# Autodesk Inventor assembly: 42146-31
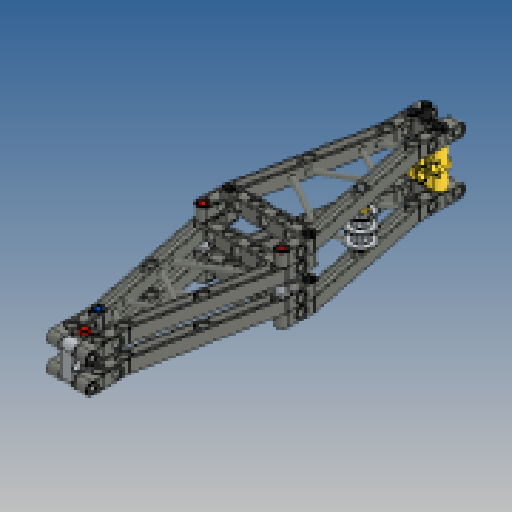
[picture p0: Inventor's stored thumbnail of the model, 512x512]
Saved by Autodesk Inventor 2025 (Build 290162010, 162A)
## iProperties
Created: 2024-12-05
Part Number: 42146-31
Material: Generisch
Document SubType Name: Assembly
Designer: hp.muther
Author: hp.muther
## Documents named in this file (15)
- D:\Inventor\Projekte\Muther\LEGO Technic\LEGO Technik - Raupenkran LR 13000 (42146)\42146-31.iam
- D:\Inventor\Projekte\Muther\LEGO Technic\LEGO Pieces\Rahmen, T-Stücke\79768-DkBluishGray.ipt
- D:\Inventor\Projekte\Muther\LEGO Technic\LEGO Pieces\Pin's\4274-Red.ipt
- D:\Inventor\Projekte\Muther\LEGO Technic\LEGO Pieces\Pin's\11214-Red.ipt
- D:\Inventor\Projekte\Muther\LEGO Technic\LEGO Pieces\Pin's\32054-LtBluishGray.ipt
- D:\Inventor\Projekte\Muther\LEGO Technic\LEGO Pieces\Pin's\2780-Black.ipt
- D:\Inventor\Projekte\Muther\LEGO Technic\LEGO Pieces\Achsen\32073-LtBluishGray.ipt
- D:\Inventor\Projekte\Muther\LEGO Technic\LEGO Pieces\Räder, Raupe\42610-LtBluishGray.ipt
- D:\Inventor\Projekte\Muther\LEGO Technic\LEGO Pieces\Pin's\6558-Blue.ipt
- D:\Inventor\Projekte\Muther\LEGO Technic\LEGO Pieces\Rund\18654-DkBluishGray.ipt
- D:\Inventor\Projekte\Muther\LEGO Technic\LEGO Pieces\Verbindungselemente\39793-Yellow.ipt
- D:\Inventor\Projekte\Muther\LEGO Technic\LEGO Pieces\Rund\4265c-Yellow.ipt
- D:\Inventor\Projekte\Muther\LEGO Technic\LEGO Pieces\Diverses\61510-LtBluishGray.ipt
- D:\Inventor\Projekte\Muther\LEGO Technic\LEGO Pieces\Pin's\77765-MediumStoneGrey.ipt
- D:\Inventor\Projekte\Muther\LEGO Technic\LEGO Pieces\Lochbalken\32523-LtBluishGray.ipt
## Components (32 placed, 14 different names)
1. 79768-DkBluishGray:1 — Einfügen:2, Einfügen:3, Einfügen:4, Einfügen:6, Einfügen:7, Einfügen:20, Einfügen:22, Einfügen:40, Einfügen:45
2. 4274-Red:1 — Einfügen:2
3. 11214-Red:1 — Einfügen:1, Passend:4
4. 32054-LtBluishGray:1 — Einfügen:1, Einfügen:7
5. 2780-Black:1 — Einfügen:3
6. 2780-Black:2 — Einfügen:4
7. 11214-Red:2
8. 32054-LtBluishGray:2 — Einfügen:6, Einfügen:26, Passend:8
9. 6558-Blue:1 — Einfügen:21, Einfügen:22
10. 18654-DkBluishGray:1 — Einfügen:21
11. 42610-LtBluishGray:4 — Einfügen:20
12. 79768-DkBluishGray:2 — Einfügen:26, Passend:4, Einfügen:34, Einfügen:43, Einfügen:44
13. 4274-Red:2
14. 2780-Black:3
15. 2780-Black:4 — Passend:7
16. 2780-Black:5
17. 2780-Black:6
18. 2780-Black:7 — Passend:6
19. 2780-Black:8
20. 39793-Yellow:1 — Einfügen:33
21. 79768-DkBluishGray:3 — Einfügen:33, Passend:6, Einfügen:34, Passend:7, Einfügen:39, Einfügen:41
22. 4265c-Yellow:1 — Einfügen:35, Fluchtend:1
23. 61510-LtBluishGray:1 — Einfügen:35, Fluchtend:1, Einfügen:37, Einfügen:38
24. 32073-LtBluishGray:3 — Einfügen:38, Einfügen:39
25. 4265c-Yellow:2
26. 61510-LtBluishGray:2 — Einfügen:37
27. 79768-DkBluishGray:4 — Einfügen:40, Passend:8, Einfügen:42
28. 2780-Black:9 — Einfügen:42
29. 2780-Black:10 — Einfügen:41
30. 77765-MediumStoneGrey:1 — Einfügen:44
31. 77765-MediumStoneGrey:2 — Einfügen:45
32. 32523-LtBluishGray:1 — Einfügen:43
## Relationships (37: Insert 31, Mate 4, Flush 2)
- Einfügen:1 [Insert]: 11214-Red:1 ↔ 32054-LtBluishGray:1
- Einfügen:2 [Insert]: 79768-DkBluishGray:1 ↔ 4274-Red:1
- Einfügen:3 [Insert]: 79768-DkBluishGray:1 ↔ 2780-Black:1
- Einfügen:4 [Insert]: 79768-DkBluishGray:1 ↔ 2780-Black:2
- [Insert]: 11214-Red:2 ↔ 32054-LtBluishGray:2
- Einfügen:6 [Insert]: 79768-DkBluishGray:1 ↔ 32054-LtBluishGray:2
- Einfügen:7 [Insert]: 79768-DkBluishGray:1 ↔ 32054-LtBluishGray:1
- Einfügen:20 [Insert]: 79768-DkBluishGray:1 ↔ 42610-LtBluishGray:4
- Einfügen:21 [Insert]: 6558-Blue:1 ↔ 18654-DkBluishGray:1
- Einfügen:22 [Insert]: 79768-DkBluishGray:1 ↔ 6558-Blue:1
- [Insert]: 79768-DkBluishGray:2 ↔ 4274-Red:2
- [Insert]: 79768-DkBluishGray:2 ↔ 2780-Black:3
- [Insert]: 79768-DkBluishGray:2 ↔ 2780-Black:4
- Einfügen:26 [Insert]: 32054-LtBluishGray:2 ↔ 79768-DkBluishGray:2
- Passend:4 [Mate]: 11214-Red:1 ↔ 79768-DkBluishGray:2
- [Insert]: 2780-Black:8 ↔ 39793-Yellow:1
- [Insert]: 2780-Black:7 ↔ 39793-Yellow:1
- [Insert]: 2780-Black:6 ↔ 39793-Yellow:1
- [Insert]: 2780-Black:5 ↔ 39793-Yellow:1
- Einfügen:33 [Insert]: 39793-Yellow:1 ↔ 79768-DkBluishGray:3
- Passend:6 [Mate]: 2780-Black:7 ↔ 79768-DkBluishGray:3
- Einfügen:34 [Insert]: 79768-DkBluishGray:2 ↔ 79768-DkBluishGray:3
- Passend:7 [Mate]: 2780-Black:4 ↔ 79768-DkBluishGray:3
- Einfügen:35 [Insert]: 4265c-Yellow:1 ↔ 61510-LtBluishGray:1
- Fluchtend:1 [Flush]: 4265c-Yellow:1 ↔ 61510-LtBluishGray:1
- [Insert]: 4265c-Yellow:2 ↔ 61510-LtBluishGray:2
- [Flush]: 4265c-Yellow:2 ↔ 61510-LtBluishGray:2
- Einfügen:37 [Insert]: 61510-LtBluishGray:1 ↔ 61510-LtBluishGray:2
- Einfügen:38 [Insert] (-28 mm): 61510-LtBluishGray:1 ↔ 32073-LtBluishGray:3
- Einfügen:39 [Insert] (-8 mm): 79768-DkBluishGray:3 ↔ 32073-LtBluishGray:3
- Einfügen:40 [Insert]: 79768-DkBluishGray:1 ↔ 79768-DkBluishGray:4
- Passend:8 [Mate]: 32054-LtBluishGray:2 ↔ 79768-DkBluishGray:4
- Einfügen:41 [Insert]: 79768-DkBluishGray:3 ↔ 2780-Black:10
- Einfügen:42 [Insert]: 79768-DkBluishGray:4 ↔ 2780-Black:9
- Einfügen:43 [Insert]: 79768-DkBluishGray:2 ↔ 32523-LtBluishGray:1
- Einfügen:44 [Insert]: 79768-DkBluishGray:2 ↔ 77765-MediumStoneGrey:1
- Einfügen:45 [Insert]: 79768-DkBluishGray:1 ↔ 77765-MediumStoneGrey:2
## Named parameters: d4_d0 = 0 mm, d26_d1 = 0 mm, d27_d2 = 0 mm, d28_d3 = 0 mm, d44_d42 = 0 mm, d45_d43 = 0 mm
